# Autodesk Inventor assembly: Assembly _ Estrutura e fechamento
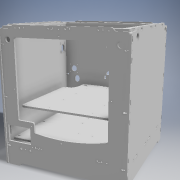
[picture p0: Inventor's stored thumbnail of the model, 180x180]
Saved by Autodesk Inventor 2016 (Build 200138000, 138)
## iProperties
Created: 2016-08-08
Part Number: Assembly _ Estrutura e fechamento
Document SubType Name: Assembly
Designer: Waldo
Author: Waldo
## Documents named in this file (8)
- C:\Users\Waldo\Documents\Inventor\RepRap\Ulticampy WALDO\Estrutura e fechamento\Assembly _ Estrutura e fechamento.iam
- C:\Users\Waldo\Documents\Inventor\RepRap\Ulticampy WALDO\Estrutura e fechamento\painel frontal.ipt
- C:\Users\Waldo\Documents\Inventor\RepRap\Ulticampy WALDO\Estrutura e fechamento\base da mesa de impressao.ipt
- C:\Users\Waldo\Documents\Inventor\RepRap\Ulticampy WALDO\Estrutura e fechamento\painel direito.ipt
- C:\Users\Waldo\Documents\Inventor\RepRap\Ulticampy WALDO\Estrutura e fechamento\painel esquerdo.ipt
- C:\Users\Waldo\Documents\Inventor\RepRap\Ulticampy WALDO\Estrutura e fechamento\painel inferior.ipt
- C:\Users\Waldo\Documents\Inventor\RepRap\Ulticampy WALDO\Estrutura e fechamento\painel superior.ipt
- C:\Users\Waldo\Documents\Inventor\RepRap\Ulticampy WALDO\Estrutura e fechamento\painel traseiro.ipt
## Components (7 placed, 7 different names)
1. painel frontal:1 — Mate:1, Mate:2, Mate:3, Mate:6, Mate:8
2. base da mesa de impressao:1 — Mate:16, Mate:17
3. painel direito:1 — Mate:7, Mate:8, Mate:9, Mate:11, Mate:14
4. painel esquerdo:1 — Mate:3, Mate:4, Mate:5, Mate:6
5. painel inferior:1 — Mate:1, Mate:2, Mate:4, Mate:5, Mate:7, Mate:9, Mate:10, Mate:12, Mate:16
6. painel superior:1 — Mate:13, Mate:14, Mate:15, Mate:17
7. painel traseiro:1 — Mate:10, Mate:11, Mate:12, Mate:13, Mate:15
## Relationships (17: Mate 17)
- Mate:1: painel frontal:1 ↔ painel inferior:1
- Mate:2: painel frontal:1 ↔ painel inferior:1
- Mate:3: painel frontal:1 ↔ painel esquerdo:1
- Mate:4: painel esquerdo:1 ↔ painel inferior:1
- Mate:5: painel esquerdo:1 ↔ painel inferior:1
- Mate:6: painel frontal:1 ↔ painel esquerdo:1
- Mate:7: painel direito:1 ↔ painel inferior:1
- Mate:8: painel frontal:1 ↔ painel direito:1
- Mate:9: painel direito:1 ↔ painel inferior:1
- Mate:10: painel inferior:1 ↔ painel traseiro:1
- Mate:11: painel direito:1 ↔ painel traseiro:1
- Mate:12: painel inferior:1 ↔ painel traseiro:1
- Mate:13: painel superior:1 ↔ painel traseiro:1
- Mate:14: painel direito:1 ↔ painel superior:1
- Mate:15: painel superior:1 ↔ painel traseiro:1
- Mate:16: base da mesa de impressao:1 ↔ painel inferior:1
- Mate:17: base da mesa de impressao:1 ↔ painel superior:1
